# Autodesk Inventor assembly: padmount_doubleservo
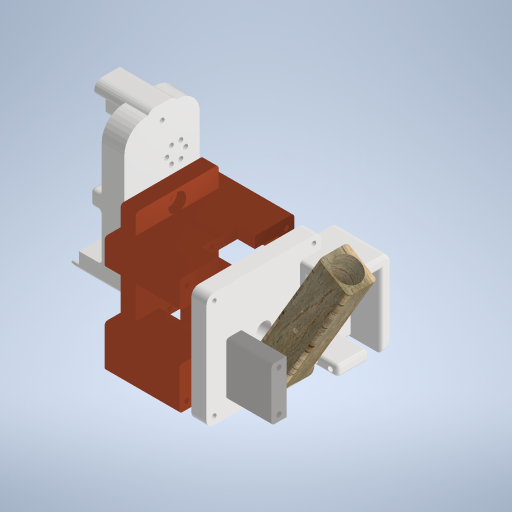
[picture p0: Inventor's stored thumbnail of the model, 512x512]
Saved by Autodesk Inventor 2023 (Build 270158000, 158)
## iProperties
Created: 2023-01-25
Part Number: padmount_doubleservo
Document SubType Name: Assembly
Designer: Hunter
Author: Hunter
## Documents named in this file (6)
- C:\Users\Hunter\Documents\ECE CAPSTONE\padmount_doubleservo.iam
- C:\Users\Hunter\Documents\ECE CAPSTONE\CAD Designs\separator_plate_alternate.ipt
- C:\Users\Hunter\Documents\ECE CAPSTONE\CAD Designs\stick_mount.ipt
- C:\Users\Hunter\Documents\ECE CAPSTONE\pulley-tensor-gt2\Slider Top 2.ipt
- C:\Users\Hunter\Documents\ECE CAPSTONE\CAD Designs\servo_horz_plate.ipt
- C:\Users\Hunter\Documents\ECE CAPSTONE\CAD Designs\servo_pressfit_plate.ipt
## Components (5 placed, 5 different names)
1. separator_plate_alternate:1 — Mate:7, Mate:8, Mate:9, Mate:23, Mate:24, Mate:25
2. stick_mount:1 — Mate:14, Mate:19
3. servo_pressfit_plate:1 — Mate:17, Mate:18, Mate:19
4. Slider Top 2:1 — Mate:7, Mate:8, Mate:9
5. servo_horz_plate:1 — Mate:14, Mate:17, Mate:18, Mate:23, Mate:24, Mate:25
## Relationships (10: Mate 10)
- Mate:7: separator_plate_alternate:1 ↔ Slider Top 2:1
- Mate:8: separator_plate_alternate:1 ↔ Slider Top 2:1
- Mate:9: separator_plate_alternate:1 ↔ Slider Top 2:1
- Mate:14 (48 mm): stick_mount:1 ↔ servo_horz_plate:1
- Mate:17: servo_pressfit_plate:1 ↔ servo_horz_plate:1
- Mate:18: servo_pressfit_plate:1 ↔ servo_horz_plate:1
- Mate:19: stick_mount:1 ↔ servo_pressfit_plate:1
- Mate:23: separator_plate_alternate:1 ↔ servo_horz_plate:1
- Mate:24: separator_plate_alternate:1 ↔ servo_horz_plate:1
- Mate:25 (8 mm): separator_plate_alternate:1 ↔ servo_horz_plate:1
